# Autodesk Inventor assembly: OBG-Gehäuse
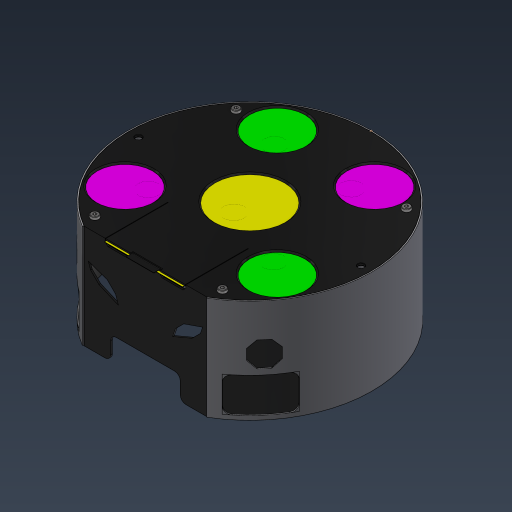
[picture p0: Inventor's stored thumbnail of the model, 512x512]
Saved by Autodesk Inventor 2023.1 (Build 271208000, 208)
## iProperties
Part Number: OBG-Gehäuse
Material: Generisch
Document SubType Name: Assembly
Designer: rYan
Mass: 129.127 g
Surface Area: 1997.42 cm^2
Volume: 130.879 cm^3
Density: 0.986618 g/cm^3
Author: rYan
## Documents named in this file (8)
- D:\TIGERsGIT\Hardware\mechanik\2024\Inventor\Robot\Case\OBG-Gehäuse.iam
- D:\TIGERsGIT\Hardware\mechanik\2024\Inventor\Robot\Case\Gehäuse Mantel.ipt
- D:\TIGERsGIT\Hardware\mechanik\2024\Inventor\Robot\Case\Gehäuse Unterplatte.ipt
- D:\TIGERsGIT\Hardware\mechanik\2024\Inventor\Purchased Parts\Papier 40mm.ipt
- D:\TIGERsGIT\Hardware\mechanik\2024\Inventor\Inhaltscenter\de-DE\DIN 7984\DIN 7984 - M3 x 5.ipt
- D:\TIGERsGIT\Hardware\mechanik\2024\Inventor\Purchased Parts\Papier Teamfarbe.ipt
- D:\TIGERsGIT\Hardware\mechanik\2024\Inventor\Robot\Case\Gehäuse Überwurf.ipt
- D:\TIGERsGIT\Hardware\mechanik\2024\Inventor\Robot\Case\Gehäuse Überwurf gespiegelt.ipt
## Components (13 placed, 7 different names)
1. Gehäuse Mantel:1 — Fluchtend:1, Passend:1, Passend:2, Einfügen:1, Passend:3, Einfügen:2, Einfügen:3, Einfügen:4, Einfügen:5, Einfügen:7, Einfügen:8, Einfügen:9, Einfügen:10, Passend:4, Passend:6, Fluchtend:3, Passend:8, Fluchtend:5
2. Gehäuse Unterplatte:1 — Einfügen:1, Passend:3
3. DIN 7984 M3 x 5:1 — Einfügen:2
4. DIN 7984 M3 x 5:2 — Einfügen:3
5. DIN 7984 M3 x 5:3 — Einfügen:5
6. DIN 7984 M3 x 5:4 — Einfügen:4
7. Papier 40mm:1 — Einfügen:9
8. Papier 40mm:2 — Einfügen:10
9. Papier 40mm:3 — Einfügen:8
10. Papier 40mm:4 — Einfügen:7
11. Papier Teamfarbe:1 — Fluchtend:2, Passend:4
12. Gehäuse Überwurf:1 — Passend:6, Passend:7, Fluchtend:3
13. Gehäuse Überwurf gespiegelt:1 — Passend:8, Fluchtend:4, Fluchtend:5
## Relationships (21: Insert 9, Mate 7, Flush 5)
- Fluchtend:1 [Flush]: Gehäuse Mantel:1
- Passend:1 [Mate]: Gehäuse Mantel:1
- Passend:2 [Mate]: Gehäuse Mantel:1
- Einfügen:1 [Insert]: Gehäuse Mantel:1 ↔ Gehäuse Unterplatte:1
- Passend:3 [Mate]: Gehäuse Mantel:1 ↔ Gehäuse Unterplatte:1
- Einfügen:2 [Insert]: Gehäuse Mantel:1 ↔ DIN 7984 M3 x 5:1
- Einfügen:3 [Insert]: Gehäuse Mantel:1 ↔ DIN 7984 M3 x 5:2
- Einfügen:4 [Insert]: Gehäuse Mantel:1 ↔ DIN 7984 M3 x 5:4
- Einfügen:5 [Insert]: Gehäuse Mantel:1 ↔ DIN 7984 M3 x 5:3
- Einfügen:7 [Insert]: Gehäuse Mantel:1 ↔ Papier 40mm:4
- Einfügen:8 [Insert]: Gehäuse Mantel:1 ↔ Papier 40mm:3
- Einfügen:9 [Insert]: Gehäuse Mantel:1 ↔ Papier 40mm:1
- Einfügen:10 [Insert]: Gehäuse Mantel:1 ↔ Papier 40mm:2
- Fluchtend:2 [Flush]: Papier Teamfarbe:1
- Passend:4 [Mate]: Gehäuse Mantel:1 ↔ Papier Teamfarbe:1
- Passend:6 [Mate]: Gehäuse Mantel:1 ↔ Gehäuse Überwurf:1
- Passend:7 [Mate]: Gehäuse Überwurf:1
- Fluchtend:3 [Flush]: Gehäuse Mantel:1 ↔ Gehäuse Überwurf:1
- Passend:8 [Mate]: Gehäuse Mantel:1 ↔ Gehäuse Überwurf gespiegelt:1
- Fluchtend:4 [Flush]: Gehäuse Überwurf gespiegelt:1
- Fluchtend:5 [Flush]: Gehäuse Mantel:1 ↔ Gehäuse Überwurf gespiegelt:1
